# Autodesk Inventor assembly: BATTERIES_CONTROLLER.brd
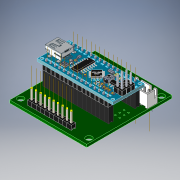
[picture p0: Inventor's stored thumbnail of the model, 180x180]
Saved by Autodesk Inventor 2022 (Build 260153000, 153)
## iProperties
Created: 2022-12-23
Part Number: BATTERIES_CONTROLLER.brd
Document SubType Name: Assembly
Designer: Ivan Petrov
Author: Ivan Petrov
## Documents named in this file (7)
- C:\Users\Ivan Petrov\Documents\GitHub\OmniBot\design\000.006 - Контроллер АКБ.iam
- C:\Users\Ivan Petrov\Documents\GitHub\OmniBot\design\000.006.001 - Плата печатная.ipt
- C:\Users\Ivan Petrov\Documents\GitHub\OmniBot\design\standart_components\smd resistors\0R.iam
- C:\Users\Ivan Petrov\Documents\GitHub\OmniBot\design\standart_components\PBS-1.ipt
- C:\Users\Ivan Petrov\Documents\GitHub\OmniBot\design\standart_components\connectrs\JST - XH - Thru (V) - 4Pin - 2.54mm.ipt
- C:\Users\Ivan Petrov\Documents\GitHub\OmniBot\design\standart_components\Arduino\Nano\Arduino Nano R3 ATmega 328P.iam
- C:\Users\Ivan Petrov\Documents\GitHub\OmniBot\design\standart_components\CONN HEADER VERT 1POS 2.54MM.ipt
## Components (59 placed, 21 different names)
1. 000.006.001 - Плата печатная — Совмещение:1, Совмещение:2, Угол:1, Совмещение:3, Совмещение:4, Совмещение:5, Совмещение:7, Совмещение:8, Угол:2
2. R1_2 [sub-assembly]
3. R2_3 [sub-assembly]
4. R3_4 [sub-assembly]
5. R4_5 [sub-assembly]
6. R5_6 [sub-assembly]
7. R6_7 [sub-assembly]
8. R7_8 [sub-assembly]
9. R8_9 [sub-assembly]
10. R9_10 [sub-assembly]
11. R10_11 [sub-assembly]
12. R11_12 [sub-assembly]
13. R12_13 [sub-assembly]
14. R13_14 [sub-assembly]
15. R14_15 [sub-assembly]
16. R15_16 [sub-assembly]
17. R16_17 [sub-assembly]
18. JST - XH - Thru (V) - 4Pin - 2.54mm:1 — Совмещение:3, Совмещение:4, Совмещение:5
19. Arduino Nano R3 ATmega 328P:1 [sub-assembly] — Заподлицо:1, Заподлицо:2, Совмещение:6
20. PBS-1:1 — Совмещение:1, Совмещение:2, Угол:1
21. PBS-1:2 — Заподлицо:1
22. PBS-1:3
23. PBS-1:4
24. PBS-1:5
25. PBS-1:6
26. PBS-1:7
27. PBS-1:8
28. PBS-1:9
29. PBS-1:10
30. PBS-1:11
31. PBS-1:12
32. PBS-1:13
33. PBS-1:14
34. PBS-1:15
35. PBS-1:16
36. PBS-1:17
37. PBS-1:18
38. PBS-1:19
39. PBS-1:20
40. PBS-1:21
41. PBS-1:22
42. PBS-1:23
43. PBS-1:24
44. PBS-1:25
45. PBS-1:26
46. PBS-1:27
47. PBS-1:28
48. PBS-1:29
49. PBS-1:30 — Заподлицо:2, Совмещение:6
50. CONN HEADER VERT 1POS 2.54MM:1 — Совмещение:7, Совмещение:8, Угол:2
51. CONN HEADER VERT 1POS 2.54MM:2
52. CONN HEADER VERT 1POS 2.54MM:3
53. CONN HEADER VERT 1POS 2.54MM:4
54. CONN HEADER VERT 1POS 2.54MM:5
55. CONN HEADER VERT 1POS 2.54MM:6
56. CONN HEADER VERT 1POS 2.54MM:7
57. CONN HEADER VERT 1POS 2.54MM:8
58. CONN HEADER VERT 1POS 2.54MM:9
59. CONN HEADER VERT 1POS 2.54MM:10
## Component patterns: (30 elements, first: PBS-1:1), (10 elements, first: CONN HEADER VERT 1POS 2.54MM:1)
## Relationships (12: Mate 8, Angle 2, Flush 2)
- Совмещение:1 [Mate]: 000.006.001 - Плата печатная ↔ PBS-1:1
- Совмещение:2 [Mate]: 000.006.001 - Плата печатная ↔ PBS-1:1
- Угол:1 [Angle] (0 deg): 000.006.001 - Плата печатная ↔ PBS-1:1
- Совмещение:3 [Mate]: 000.006.001 - Плата печатная ↔ JST - XH - Thru (V) - 4Pin - 2.54mm:1
- Совмещение:4 [Mate]: 000.006.001 - Плата печатная ↔ JST - XH - Thru (V) - 4Pin - 2.54mm:1
- Совмещение:5 [Mate]: 000.006.001 - Плата печатная ↔ JST - XH - Thru (V) - 4Pin - 2.54mm:1
- Заподлицо:1 [Flush]: Arduino Nano R3 ATmega 328P:1 ↔ PBS-1:2
- Заподлицо:2 [Flush]: Arduino Nano R3 ATmega 328P:1 ↔ PBS-1:30
- Совмещение:6 [Mate]: Arduino Nano R3 ATmega 328P:1 ↔ PBS-1:30
- Совмещение:7 [Mate]: 000.006.001 - Плата печатная ↔ CONN HEADER VERT 1POS 2.54MM:1
- Совмещение:8 [Mate]: 000.006.001 - Плата печатная ↔ CONN HEADER VERT 1POS 2.54MM:1
- Угол:2 [Angle] (0 deg): 000.006.001 - Плата печатная ↔ CONN HEADER VERT 1POS 2.54MM:1
